# Autodesk Inventor assembly: Spine test
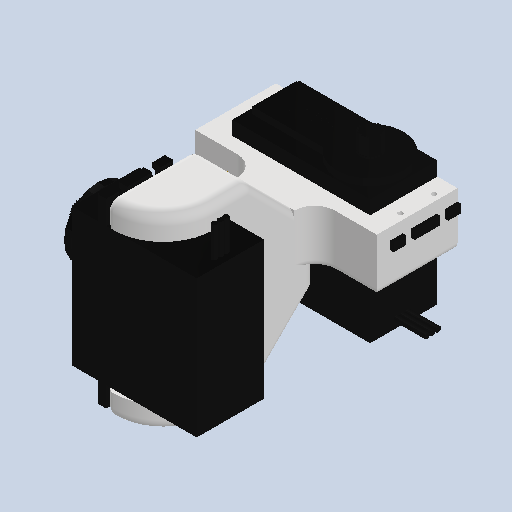
[picture p0: Inventor's stored thumbnail of the model, 512x512]
Saved by Autodesk Inventor 2022 (Build 260153000, 153)
## iProperties
Created: 2022-05-09
Part Number: Spine test
Document SubType Name: Assembly
Designer: dirks
Author: dirks
## Documents named in this file (3)
- C:\Users\dirks\Arny-de-humanoid-robot\Parts\Tests\Spine test.iam
- C:\Users\dirks\Arny-de-humanoid-robot\Parts\Spine head servo connector.ipt
- C:\Users\dirks\Arny-de-humanoid-robot\Parts\Imported Components\SERVO motor\Servo MOtor.ipt
## Components (3 placed, 2 different names)
1. Servo MOtor:1
2. Spine head servo connector:1 — Mate:1, Mate:3, Mate:4
3. Servo MOtor:2 — Mate:1, Mate:3, Mate:4
## Relationships (3: Mate 3)
- Mate:1: Spine head servo connector:1 ↔ Servo MOtor:2
- Mate:3: Spine head servo connector:1 ↔ Servo MOtor:2
- Mate:4: Spine head servo connector:1 ↔ Servo MOtor:2
